# Autodesk Inventor assembly: xt90
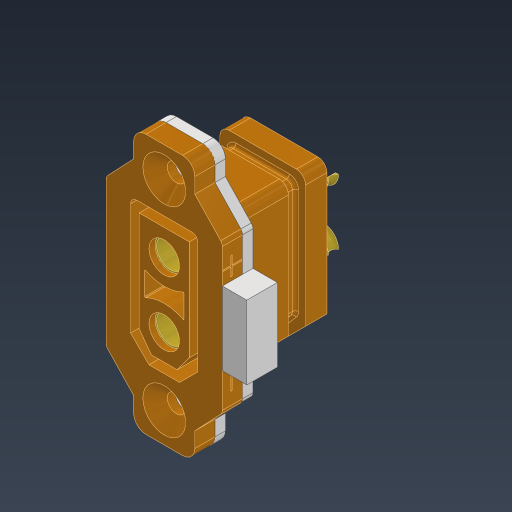
[picture p0: Inventor's stored thumbnail of the model, 512x512]
Saved by Autodesk Inventor 2023 (Build 270158000, 158)
## iProperties
Created: 2024-10-09
Part Number: xt90
Description: FreeCAD Model
Document SubType Name: Assembly
Designer: szymo
Authority: Unknown
Sending System: Ondsel
Preprocessor: Open CASCADE STEP processor 7.7
Title: Open CASCADE Shape Model
Author: Author
## Documents named in this file (5)
- D:\tech\diy\e-skateboard\projekcik-inventor\xt90.iam
- D:\tech\diy\e-skateboard\projekcik-inventor\pino-.ipt
- D:\tech\diy\e-skateboard\projekcik-inventor\pino+.ipt
- D:\tech\diy\e-skateboard\projekcik-inventor\Corpo.ipt
- D:\tech\diy\e-skateboard\projekcik-inventor\4.ipt
## Components (4 placed, 4 different names)
1. 1
2. 2
3. 3 — Flush:1, Flush:2
4. 4:1 — Flush:1, Flush:2
## Relationships (2: Flush 2)
- Flush:1: 3 ↔ 4:1
- Flush:2: 3 ↔ 4:1
